# Autodesk Inventor assembly: Assembly1
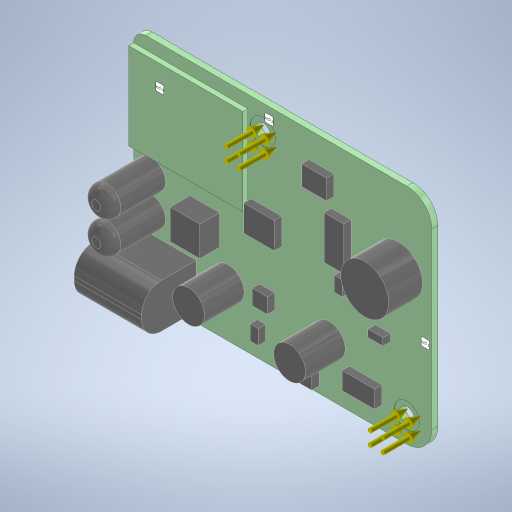
[picture p0: Inventor's stored thumbnail of the model, 512x512]
Saved by Autodesk Inventor 2023 (Build 270158000, 158)
## iProperties
Created: 2024-10-12
Part Number: Assembly1
Document SubType Name: Assembly
Designer: noname
Author: noname
## Documents named in this file (9)
- C:\Users\noname\Documents\GitHub\Seismometer-esp32\Case\Assembly1.iam
- C:\Users\noname\Documents\GitHub\Seismometer-esp32\Case\Part1.ipt
- C:\Users\noname\Documents\GitHub\Seismometer-esp32\Case\Part2.ipt
- C:\Users\noname\Documents\GitHub\Seismometer-esp32\Case\Assembly1\AIP\FEA\eulmvy44g.fins
- C:\Users\noname\Documents\GitHub\Seismometer-esp32\Case\Assembly1\AIP\FEA\eulmvy44g.fsat
- C:\Users\noname\Documents\GitHub\Seismometer-esp32\Case\Assembly1\AIP\FEA\eulmvy44g.ftes
- C:\Users\noname\Documents\GitHub\Seismometer-esp32\Case\Assembly1\AIP\FEA\eulmvy44g.fwiz
- C:\Users\noname\Documents\GitHub\Seismometer-esp32\Case\Assembly1\AIP\FEA\eulmvy45c.fmsh
- C:\Users\noname\Documents\GitHub\Seismometer-esp32\Case\Assembly1\AIP\FEA\eulmvy45d.fres
## Components (2 placed, 2 different names)
1. Part1:1 — Mate:1, Flush:1, Flush:2
2. Part2:1 — Mate:1, Flush:1, Flush:2
## Relationships (3: Flush 2, Mate 1)
- Mate:1: Part1:1 ↔ Part2:1
- Flush:1 (-1 mm): Part1:1 ↔ Part2:1
- Flush:2 (2 mm): Part1:1 ↔ Part2:1
## Named parameters: sa_0 = 50000, sa_f1 = 450.454
note: some values were not read from the file. Shown as the stored number, unit unknown: "sa_0", "sa_f1".
